# Autodesk Inventor assembly: speaker stand assembly
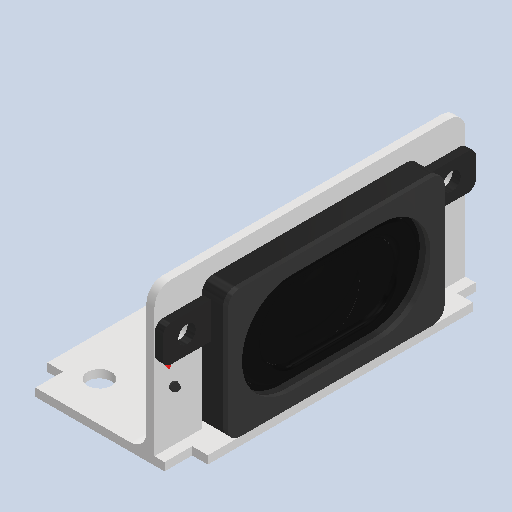
[picture p0: Inventor's stored thumbnail of the model, 512x512]
Saved by Autodesk Inventor 2022.2 (Build 262287000, 287)
## iProperties
Created: 2022-02-22
Part Number: speaker stand assembly
Document SubType Name: Assembly
Designer: ONG
Author: ONG
## Documents named in this file (3)
- C:\Users\ONG\Documents\INVENTOR DESIGN\音箱\speaker stand assembly.iam
- C:\Users\ONG\Downloads\Small-Speaker-2715.iam
- C:\Users\ONG\Documents\INVENTOR DESIGN\音箱\spekaer cover.ipt
## Components (2 placed, 2 different names)
1. Small-Speaker-2715:1 [sub-assembly] — Mate:1, Flush:1, Flush:2
2. spekaer cover:1 — Mate:1, Flush:1, Flush:2
## Relationships (3: Flush 2, Mate 1)
- Mate:1: Small-Speaker-2715:1 ↔ spekaer cover:1
- Flush:1: Small-Speaker-2715:1 ↔ spekaer cover:1
- Flush:2 (2.5 mm): Small-Speaker-2715:1 ↔ spekaer cover:1
